# Autodesk Inventor assembly: GearAssembly
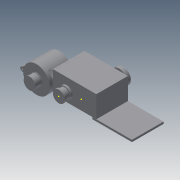
[picture p0: Inventor's stored thumbnail of the model, 180x180]
Saved by Autodesk Inventor 2015 (Build 190159000, 159)
## iProperties
Created: 2014-08-31
Part Number: GearAssembly
Document SubType Name: Assembly
Designer: shohei
Author: shohei
## Documents named in this file (11)
- C:\Users\shohei\Documents\Inventor\FufuPounderGeared\GearAssembly_rev1.iam
- C:\Users\shohei\Documents\Inventor\FufuPounderGeared\alternator.ipt
- C:\Users\shohei\Documents\Inventor\FufuPounderGeared\schaft1.ipt
- C:\Users\shohei\Documents\Inventor\FufuPounderGeared\Spur Gears1.iam
- C:\Users\shohei\Documents\Inventor\FufuPounderGeared\Spur Gears2.iam
- C:\Users\shohei\Documents\Inventor\FufuPounderGeared\shaft_cover.ipt
- C:\Users\shohei\Documents\Inventor\FufuPounderGeared\gearSupport.ipt
- C:\Users\shohei\Documents\Inventor\FufuPounderGeared\boxsupport.ipt
- C:\Users\shohei\Documents\Inventor\FufuPounderGeared\boxsupport2.ipt
- C:\Users\shohei\Documents\Inventor\FufuPounderGeared\pulley.ipt
- C:\Users\shohei\Documents\Inventor\FufuPounderGeared\flywheel.ipt
## Components (23 placed, 9 different names)
1. alternator:1 — Mate:8
2. schaft1:1 — Mate:2, Mate:4, Rotational:8, Rotational:24, Rotational:27
3. schaft1:2 — Mate:4, Mate:6, Rotational:12, Rotational:25, Rotational:26
4. Spur Gears:1 [sub-assembly] — Rotational:8, Rotation:4, Rotational:13, Angle:4, Rotational:22, Angle:7, Angle:9
5. Spur Gears:3 [sub-assembly] — Rotational:5, Angle:2, Rotational:12, Rotation:4
6. Spur Gears:4 [sub-assembly] — Angle:3, Rotation:6, Rotational:15, Rotational:17
7. Spur Gears:5 [sub-assembly] — Rotational:5, Angle:2, Rotation:5, Rotational:14
8. Spur Gears:6 [sub-assembly] — Rotational:17, Rotation:7, Rotational:18, Angle:6
9. Spur Gears:7 [sub-assembly] — Rotational:13, Rotation:5, Angle:3, Rotational:15
10. Spur Gears:8 [sub-assembly] — Rotational:18, Angle:6, Rotation:8
11. Spur Gears:9 [sub-assembly] — Rotational:16, Angle:5, Rotation:7, Rotational:19
12. Spur Gears:10 [sub-assembly] — Rotational:14, Rotation:6, Rotational:16, Angle:5
13. shaft_cover:1 — Rotational:25, Mate:10, Flush:3, Flush:4, Mate:12, Flush:9
14. Spur Gears:11 [sub-assembly] — Rotational:19, Rotation:8, Rotational:23, Angle:8, Angle:10
15. shaft_cover:2 — Rotational:24, Flush:1, Mate:9, Flush:2, Mate:11, Flush:6, Flush:8, Mate:13
16. gearSupport:1 — Rotational:22, Angle:7
17. gearSupport:2 — Rotational:23, Angle:8
18. boxsupport:1 — Flush:1, Mate:9, Flush:2, Mate:10, Flush:3, Flush:4, Flush:5, Flush:7
19. boxsupport:2 — Mate:13, Flush:9
20. boxsupport2:1 — Mate:12, Flush:7, Flush:8
21. boxsupport2:2 — Mate:11, Flush:5, Flush:6
22. pulley:1 — Rotational:27, Angle:9
23. flywheel:1 — Rotational:26, Angle:10
## Relationships (48: RevoluteJoint 16, Mate 9, Angle 9, Flush 9, RelateRotation 5)
- Mate:2: schaft1:1
- Mate:4 (70 mm): schaft1:1 ↔ schaft1:2
- Mate:6: schaft1:2
- Rotational:5 [RevoluteJoint]: Spur Gears:3 ↔ Spur Gears:5
- Angle:2 (0 deg): Spur Gears:3 ↔ Spur Gears:5
- Rotational:8 [RevoluteJoint] (-75 mm): schaft1:1 ↔ Spur Gears:1
- Rotational:12 [RevoluteJoint] (-30 mm): schaft1:2 ↔ Spur Gears:3
- Rotation:4 [RelateRotation] (0.625 ul): Spur Gears:1 ↔ Spur Gears:3
- Rotational:13 [RevoluteJoint]: Spur Gears:1 ↔ Spur Gears:7
- Rotation:5 [RelateRotation] (1.6 ul): Spur Gears:5 ↔ Spur Gears:7
- Angle:3 (0 deg): Spur Gears:4 ↔ Spur Gears:7
- Angle:4 (227 deg): Spur Gears:1
- Rotational:14 [RevoluteJoint]: Spur Gears:5 ↔ Spur Gears:10
- Rotation:6 [RelateRotation] (1.6 ul): Spur Gears:4 ↔ Spur Gears:10
- Rotational:15 [RevoluteJoint]: Spur Gears:4 ↔ Spur Gears:7
- Rotational:16 [RevoluteJoint]: Spur Gears:9 ↔ Spur Gears:10
- Angle:5 (0 deg): Spur Gears:9 ↔ Spur Gears:10
- Rotational:17 [RevoluteJoint]: Spur Gears:4 ↔ Spur Gears:6
- Rotation:7 [RelateRotation] (0.625 ul): Spur Gears:6 ↔ Spur Gears:9
- Rotational:18 [RevoluteJoint]: Spur Gears:6 ↔ Spur Gears:8
- Angle:6 (0 deg): Spur Gears:6 ↔ Spur Gears:8
- Rotational:19 [RevoluteJoint]: Spur Gears:9 ↔ Spur Gears:11
- Rotation:8 [RelateRotation] (1.6 ul): Spur Gears:8 ↔ Spur Gears:11
- Rotational:22 [RevoluteJoint]: Spur Gears:1 ↔ gearSupport:1
- Rotational:23 [RevoluteJoint]: Spur Gears:11 ↔ gearSupport:2
- Mate:8: alternator:1
- Angle:7 (0 deg): Spur Gears:1 ↔ gearSupport:1
- Angle:8 (0 deg): Spur Gears:11 ↔ gearSupport:2
- Rotational:24 [RevoluteJoint] (-5 mm): schaft1:1 ↔ shaft_cover:2
- Rotational:25 [RevoluteJoint]: schaft1:2 ↔ shaft_cover:1
- Flush:1: shaft_cover:2 ↔ boxsupport:1
- Mate:9: shaft_cover:2 ↔ boxsupport:1
- Flush:2: shaft_cover:2 ↔ boxsupport:1
- Mate:10: shaft_cover:1 ↔ boxsupport:1
- Flush:3: shaft_cover:1 ↔ boxsupport:1
- Flush:4: shaft_cover:1 ↔ boxsupport:1
- Mate:11: shaft_cover:2 ↔ boxsupport2:2
- Flush:5: boxsupport:1 ↔ boxsupport2:2
- Flush:6: shaft_cover:2 ↔ boxsupport2:2
- Mate:12: shaft_cover:1 ↔ boxsupport2:1
- Flush:7: boxsupport:1 ↔ boxsupport2:1
- Flush:8: shaft_cover:2 ↔ boxsupport2:1
- Mate:13: shaft_cover:2 ↔ boxsupport:2
- Flush:9: shaft_cover:1 ↔ boxsupport:2
- Rotational:26 [RevoluteJoint]: schaft1:2 ↔ flywheel:1
- Rotational:27 [RevoluteJoint]: schaft1:1 ↔ pulley:1
- Angle:9 (0 deg): Spur Gears:1 ↔ pulley:1
- Angle:10 (0 deg): Spur Gears:11 ↔ flywheel:1
